# Autodesk Inventor assembly: Stewart-Platform-Außenanordnung
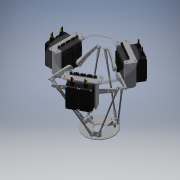
[picture p0: Inventor's stored thumbnail of the model, 180x180]
Saved by Autodesk Inventor 2018.2 (Build 222227000, 227)
## iProperties
Created: 2018-02-17
Part Number: Stewart-Platform-Außenanordnung
Material: Generisch
Document SubType Name: Assembly
Designer: JochenAlt
Author: JochenAlt
## Documents named in this file (6)
- D:\Projects\PrivateDancer\CAD\Stewart-Platform.iam
- D:\Projects\PrivateDancer\CAD\Servo-Holder.iam
- D:\Projects\PrivateDancer\CAD\Stewart-Platform-Base.ipt
- D:\Projects\PrivateDancer\CAD\Ball-Joint-Rod.iam
- D:\Projects\PrivateDancer\CAD\Servo-Arm-38mm-Ball-Joint.iam
- D:\Projects\PrivateDancer\CAD\Stewart-Plate.iam
## Components (17 placed, 5 different names)
1. ServoHolder:1 [sub-assembly] — Passend:3, Passend:4, Passend:7, Passend:8, Passend:10, Passend:11
2. ServoHolder:2 [sub-assembly] — Passend:5, Passend:6, Passend:19, Passend:20, Passend:21, Passend:22
3. ServoHolder:3 [sub-assembly] — Passend:1, Passend:2, Passend:13, Passend:14, Passend:15, Passend:16
4. Stewart-Platform-Base:1 — Passend:1, Passend:2, Passend:3, Passend:4, Passend:5, Passend:6
5. Ball Joint Rod:1 [sub-assembly] — Passend:12, Passend:29
6. Ball Joint Rod:2 [sub-assembly] — Passend:9, Passend:30
7. Servo Lever ball joint:1 [sub-assembly] — Passend:10, Passend:11, Passend:12
8. Servo Lever ball joint:2 [sub-assembly] — Passend:7, Passend:8, Passend:9
9. Servo Lever ball joint:3 [sub-assembly] — Passend:13, Passend:16, Passend:18
10. Servo Lever ball joint:4 [sub-assembly] — Passend:14, Passend:15, Passend:17
11. Servo Lever ball joint:5 [sub-assembly] — Passend:19, Passend:22, Passend:24
12. Servo Lever ball joint:6 [sub-assembly] — Passend:20, Passend:21, Passend:23
13. Ball Joint Rod:3 [sub-assembly] — Passend:17, Passend:26
14. Ball Joint Rod:4 [sub-assembly] — Passend:18, Passend:25
15. Ball Joint Rod:5 [sub-assembly] — Passend:24, Passend:28
16. Ball Joint Rod:6 [sub-assembly] — Passend:23, Passend:27
17. Stewart-Plate:1 [sub-assembly] — Passend:25, Passend:26, Passend:27, Passend:28, Passend:29, Passend:30
## Relationships (30: Mate 30)
- Passend:1 [Mate]: ServoHolder:3 ↔ Stewart-Platform-Base:1
- Passend:2 [Mate]: ServoHolder:3 ↔ Stewart-Platform-Base:1
- Passend:3 [Mate]: ServoHolder:1 ↔ Stewart-Platform-Base:1
- Passend:4 [Mate]: ServoHolder:1 ↔ Stewart-Platform-Base:1
- Passend:5 [Mate]: ServoHolder:2 ↔ Stewart-Platform-Base:1
- Passend:6 [Mate]: ServoHolder:2 ↔ Stewart-Platform-Base:1
- Passend:7 [Mate]: ServoHolder:1 ↔ Servo Lever ball joint:2
- Passend:8 [Mate]: ServoHolder:1 ↔ Servo Lever ball joint:2
- Passend:9 [Mate]: Ball Joint Rod:2 ↔ Servo Lever ball joint:2
- Passend:10 [Mate]: ServoHolder:1 ↔ Servo Lever ball joint:1
- Passend:11 [Mate]: ServoHolder:1 ↔ Servo Lever ball joint:1
- Passend:12 [Mate]: Ball Joint Rod:1 ↔ Servo Lever ball joint:1
- Passend:13 [Mate]: ServoHolder:3 ↔ Servo Lever ball joint:3
- Passend:14 [Mate]: ServoHolder:3 ↔ Servo Lever ball joint:4
- Passend:15 [Mate]: ServoHolder:3 ↔ Servo Lever ball joint:4
- Passend:16 [Mate]: ServoHolder:3 ↔ Servo Lever ball joint:3
- Passend:17 [Mate]: Servo Lever ball joint:4 ↔ Ball Joint Rod:3
- Passend:18 [Mate]: Servo Lever ball joint:3 ↔ Ball Joint Rod:4
- Passend:19 [Mate]: ServoHolder:2 ↔ Servo Lever ball joint:5
- Passend:20 [Mate]: ServoHolder:2 ↔ Servo Lever ball joint:6
- Passend:21 [Mate]: ServoHolder:2 ↔ Servo Lever ball joint:6
- Passend:22 [Mate]: ServoHolder:2 ↔ Servo Lever ball joint:5
- Passend:23 [Mate]: Servo Lever ball joint:6 ↔ Ball Joint Rod:6
- Passend:24 [Mate]: Servo Lever ball joint:5 ↔ Ball Joint Rod:5
- Passend:25 [Mate]: Ball Joint Rod:4 ↔ Stewart-Plate:1
- Passend:26 [Mate]: Ball Joint Rod:3 ↔ Stewart-Plate:1
- Passend:27 [Mate]: Ball Joint Rod:6 ↔ Stewart-Plate:1
- Passend:28 [Mate]: Ball Joint Rod:5 ↔ Stewart-Plate:1
- Passend:29 [Mate]: Ball Joint Rod:1 ↔ Stewart-Plate:1
- Passend:30 [Mate]: Ball Joint Rod:2 ↔ Stewart-Plate:1
